# Autodesk Inventor assembly: hoops_sml_med_lrg
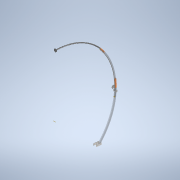
[picture p0: Inventor's stored thumbnail of the model, 180x180]
Saved by Autodesk Inventor 2021 (Build 250183000, 183)
## iProperties
Created: 2021-05-05
Part Number: hoops_sml_med_lrg
Document SubType Name: Assembly
Mass: 12206.6 g
Surface Area: 10778.2 cm^2
Volume: 1775.93 cm^3
Density: 6.87339 g/cm^3
## Documents named in this file (12)
- C:\Users\ocon0143\OneDrive - Flinders\Advn Mech Design Shared\6_Development\2_Design\inventor\hoop_slider\hoops_sml_med_lrg.iam
- C:\Users\ocon0143\OneDrive - Flinders\Advn Mech Design Shared\6_Development\2_Design\inventor\hoop_slider\large_hoop.ipt
- C:\Users\ocon0143\OneDrive - Flinders\Advn Mech Design Shared\6_Development\2_Design\inventor\hoop_slider\medium_hoop.ipt
- C:\Users\ocon0143\OneDrive - Flinders\Advn Mech Design Shared\6_Development\2_Design\inventor\rack_pinion\pinion.ipt
- C:\Users\ocon0143\OneDrive - Flinders\Advn Mech Design Shared\6_Development\2_Design\inventor\hoop_slider\small_hoop.ipt
- C:\Users\ocon0143\OneDrive - Flinders\Advn Mech Design Shared\6_Development\2_Design\inventor\rack_pinion\tooth.ipt
- C:\Users\ocon0143\OneDrive - Flinders\Advn Mech Design Shared\6_Development\2_Design\inventor\rack_pinion\large_bearings.ipt
- C:\Users\ocon0143\OneDrive - Flinders\Advn Mech Design Shared\6_Development\2_Design\inventor\rack_pinion\medium_bearings.ipt
- C:\Users\ocon0143\OneDrive - Flinders\Advn Mech Design Shared\6_Development\2_Design\inventor\rack_pinion\medium_pulley.ipt
- C:\Users\ocon0143\OneDrive - Flinders\Advn Mech Design Shared\6_Development\2_Design\inventor\hoop_slider\hoop_tab.ipt
- C:\Users\ocon0143\OneDrive - Flinders\Advn Mech Design Shared\6_Development\2_Design\inventor\hoop_slider\hoop_tab_extender.ipt
- C:\Users\ocon0143\OneDrive - Flinders\Advn Mech Design Shared\6_Development\2_Design\inventor\params.xlsx
## Components (90 placed, 10 different names)
1. large_hoop:1 — Mate:1, Flush:1, Flush:12, Flush:16, Mate:16, Mate:21, Mate:30, Tangent:1, Tangent:2, Angle:4, Angle:5, Mate:31, Mate:32, Tangent:4, Tangent:5
2. medium_hoop:1 — Mate:2, Flush:2, Mate:4, Flush:8, Mate:6, Mate:7, Mate:14, Mate:15, Mate:33
3. pinion:1 — Flush:6, Mate:34, Flush:18, Mate:35
4. small_hoop:1 — Mate:3, Flush:7
5. large_bearings:1 — Mate:6, Flush:12, Mate:16
6. medium_bearings:1 — Flush:13, Mate:7, Mate:15
7. medium_pulley:1 — Mate:11, Mate:14
8. hoop_tab:1 — Mate:21, Mate:26, Mate:29, Tangent:2, Angle:5
9. hoop_tab:2 — Mate:24, Angle:2, Mate:28, Mate:30, Tangent:1
10. hoop_tab_extender:1 — Mate:24, Angle:2, Mate:28, Flush:17, Angle:7
11. hoop_tab_extender:2 — Mate:26, Mate:29, Flush:17, Angle:4, Angle:8
12. hoop_tab:3 — Mate:31, Angle:8, Tangent:5
13. hoop_tab:4 — Mate:32, Angle:7, Tangent:4
14. tooth:1 — Mate:4, Flush:8, Mate:33
15. tooth:2
16. tooth:3
17. tooth:4
18. tooth:5
19. tooth:6
20. tooth:7
21. tooth:8
22. tooth:9
23. tooth:10
24. tooth:11
25. tooth:12
26. tooth:13
27. tooth:14
28. tooth:15
29. tooth:16
30. tooth:17
31. tooth:18
32. tooth:19
33. tooth:20
34. tooth:21
35. tooth:22
36. tooth:23
37. tooth:24
38. tooth:25
39. tooth:26
40. tooth:27
41. tooth:28
42. tooth:29
43. tooth:30
44. tooth:31
45. tooth:32
46. tooth:33
47. tooth:34
48. tooth:35
49. tooth:36
50. tooth:37
51. tooth:38
52. tooth:39
53. tooth:40
54. tooth:41
55. tooth:42
56. tooth:43
57. tooth:44
58. tooth:45
59. tooth:46
60. tooth:47
61. tooth:48
62. tooth:49
63. tooth:50
64. tooth:51
65. tooth:52
66. tooth:53
67. tooth:54
68. tooth:55
69. tooth:56
70. tooth:57
71. tooth:58
72. tooth:59
73. tooth:60
74. tooth:61
75. tooth:62
76. tooth:63
77. tooth:64
78. tooth:65 — Mate:34, Flush:18, Mate:35
79. tooth:66
80. tooth:67
81. tooth:68
82. tooth:69
83. tooth:70
84. tooth:71
85. tooth:72
86. tooth:73
87. tooth:74
88. tooth:75
89. tooth:76
90. tooth:77
## Component patterns: (64 elements, first: tooth:1), (13 elements, first: tooth:65)
## Relationships (41: Mate 21, Flush 11, Angle 5, Tangent 4)
- Mate:1: large_hoop:1
- Mate:2: medium_hoop:1
- Flush:1: large_hoop:1
- Flush:2: medium_hoop:1
- Flush:6: pinion:1
- Mate:3: small_hoop:1
- Flush:7: small_hoop:1
- Mate:4: medium_hoop:1 ↔ tooth:1
- Flush:8: medium_hoop:1 ↔ tooth:1
- Mate:6: medium_hoop:1 ↔ large_bearings:1
- Flush:12: large_hoop:1 ↔ large_bearings:1
- Flush:13: medium_bearings:1
- Mate:7: medium_hoop:1 ↔ medium_bearings:1
- Mate:11: medium_pulley:1
- Flush:14
- Mate:14: medium_hoop:1 ↔ medium_pulley:1
- Mate:15: medium_hoop:1 ↔ medium_bearings:1
- Flush:16: large_hoop:1
- Mate:16: large_hoop:1 ↔ large_bearings:1
- Mate:21: large_hoop:1 ↔ hoop_tab:1
- Mate:24: hoop_tab:2 ↔ hoop_tab_extender:1
- Mate:26: hoop_tab:1 ↔ hoop_tab_extender:2
- Angle:2 (0 deg): hoop_tab:2 ↔ hoop_tab_extender:1
- Mate:28: hoop_tab:2 ↔ hoop_tab_extender:1
- Mate:29: hoop_tab:1 ↔ hoop_tab_extender:2
- Mate:30: large_hoop:1 ↔ hoop_tab:2
- Tangent:1: large_hoop:1 ↔ hoop_tab:2
- Tangent:2: large_hoop:1 ↔ hoop_tab:1
- Flush:17: hoop_tab_extender:1 ↔ hoop_tab_extender:2
- Angle:4 (-6 deg): large_hoop:1 ↔ hoop_tab_extender:2
- Angle:5 (0 deg): large_hoop:1 ↔ hoop_tab:1
- Mate:31: large_hoop:1 ↔ hoop_tab:3
- Mate:32: large_hoop:1 ↔ hoop_tab:4
- Angle:7 (0 deg): hoop_tab_extender:1 ↔ hoop_tab:4
- Tangent:4: large_hoop:1 ↔ hoop_tab:4
- Angle:8 (0 deg): hoop_tab_extender:2 ↔ hoop_tab:3
- Tangent:5: large_hoop:1 ↔ hoop_tab:3
- Mate:33: medium_hoop:1 ↔ tooth:1
- Mate:34: pinion:1 ↔ tooth:65
- Flush:18: pinion:1 ↔ tooth:65
- Mate:35 (6 mm): pinion:1 ↔ tooth:65
## Named parameters: testLength = 1000 mm, testWidth = 1500 mm, testHeight = 1700 mm, rack_tooth_thickness = 5 mm, rack_tooth_face_widh = 10 mm, rack_tooth_addendum = 5 mm, rack_tooth_dedendum = 5 mm, hoop_radius_large = 3300 mm, hoop_width_large = 51 mm, hoop_thickness_large = 4 mm, hoop_width_medium = 33.7 mm, hoop_thickness_medium = 3.2 mm, hoop_width_small = 25.4 mm, hoop_thickness_small = 2 mm, hoop_height_large = 450 mm, hoop_height_medium = 450 mm, hoop_height_small = 600 mm, hoop_length_large = 200 mm, hoop_length_medium = 700 mm, hoop_length_small = 700 mm, cover_width_main = 1600 mm, cover_height_main = 900 mm, cover_length_main = 2200 mm, cover_shell_thickness = 10 mm, cover_base_thickness = 10 mm, cover_mountHole_diameter = 10 mm, cover_mountHole_xSpacing = 900 mm, cover_mountHole_ySpacing = 550 mm, cover_side_thickness = 20 mm, cover_side_openSize = 1400 mm, hoop_bearing_length = 5 deg, hoop_cable_diam = 5 mm, hoop_cable_pulley_diam = 22 mm, secure_arm_length = 300 mm, secure_arm_radii = 9 mm, secure_arm_hold_length = 50 mm, secure_arm_hold_thickness = 30 mm, secure_arm_thickness = 30 mm, secure_arm_angle = 35 deg, support_frame_squareBarThickness = 5 mm, support_frame_squareBarDimension = 50 mm, support_frame_squareBarFillet = 2 mm, support_baseClamp_platformThickness = 15 mm, support_baseClamp_sleeve_hole2Height = 100 mm, support_baseClamp_platformWidthBuffer = 0 mm, support_baseClamp_sleeveThickness = 20 mm, support_baseClamp_platformLengthBuffer = 35 mm, support_baseClamp_sleeve_hole1Height = 50 mm, support_frame_length = 500 mm, support_frame_endHoleBuffer = 45 mm, support_frame_clampHoleSpacing = 100 mm, support_frame_clampHoleDiameter = 10 mm, support_baseClamp_thickness = 8 mm, support_baseClamp_sleeveSweepTerminationAngle = 55 deg, support_baseClamp_sleeveHoleDiameter = 12 mm, support_baseClamp_lengthBuffer = 40 mm, hoop_offset_x = 660 mm, hoop_angle_z = 45 deg, hoop_tabs_hole = 12 mm, hoop_tabs_width = 50 mm, hoop_tabs_thickness = 6 mm, wheelchair_deployed_length = 1067 mm, wheelchair_deployed_height = 914 mm, wheelchair_wheel_radius = 240 mm, wheelchair_deployed_width = 635 mm, wheelchair_folded_width = 280 mm, sm_varx_member_tolerance = 0 mm, sm_varx_x = 100 mm, sm_varx_squareBarThickness = 2.5 mm, sm_varx_z = 160 mm, sm_varx_pinPlate_aspectRatio = 2, sm_varx_x_arms = 50 mm, sm_varx_pinPlate_holeDiameter = 5 mm, sm_varx_pinPlate_thickness = 5 mm, sm_varx_y = 250 mm, sm_varx_squareBarDimension = 30 mm, hoop_bushing12_radialInterference = 0 mm, hoop_bushing23_radialInterference = 0 mm, hoop_bushing23_od = 27.3 mm, hoop_bushing12_od = 43 mm, wheelchatir_pos_deploy_angle_0 = 65 deg, wheelchatir_pos_store_angle_0 = 90 deg, wheelchatir_pos_deploy_angle_1 = 20 deg, wheelchatir_pos_store_angle_1 = 20 deg, hoop_bushing12_thickness = 9.3 mm, hoop_bushing23_thickness = 1.9 mm
